# Autodesk Inventor assembly: Hoja Oculta
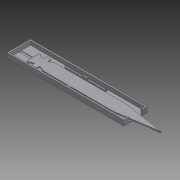
[picture p0: Inventor's stored thumbnail of the model, 180x180]
Saved by Autodesk Inventor 2011 (Build 150239000, 239)
## iProperties
Created: 2014-08-14
Part Number: Hoja Oculta
Document SubType Name: Assembly
Designer: amatiasq
Author: amatiasq
## Documents named in this file (3)
- C:\Users\amatiasq\Documents\GitHub\3D\Hoja Oculta Inventor\Piezas\Hoja Oculta.iam
- C:\Users\amatiasq\Documents\GitHub\3D\Hoja Oculta Inventor\Piezas\Base.ipt
- C:\Users\amatiasq\Documents\GitHub\3D\Hoja Oculta Inventor\Piezas\Hoja.ipt
## Components (2 placed, 2 different names)
1. Base:1 — Coincidencia:1
2. Hoja:1 — Coincidencia:1
## Relationships (1: Mate 1)
- Coincidencia:1 [Mate] (0.3 mm): Base:1 ↔ Hoja:1
